# Autodesk Inventor assembly: AssemblyGefreesdBasev2
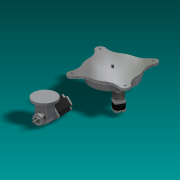
[picture p0: Inventor's stored thumbnail of the model, 180x180]
Saved by Autodesk Inventor 2020.2 (Build 242310000, 310)
## iProperties
Created: 2020-05-18
Part Number: AssemblyGefreesdBasev2
Document SubType Name: Assembly
Designer: Svend
Author: Svend
## Documents named in this file (14)
- C:\Users\Svend\OneDrive\Documents\GitHub\BeerMinder\3D-model\Base (Axis 1)\gefreesd\AssemblyGefreesdBasev2.iam
- C:\Users\Svend\OneDrive\Documents\GitHub\BeerMinder\3D-model\subAssembly\Nema17MetGearbox.iam
- C:\Users\Svend\OneDrive\Documents\GitHub\BeerMinder\3D-model\gearbox\afstandsplaatje.ipt
- C:\Users\Svend\OneDrive\Documents\GitHub\BeerMinder\3D-model\bearings\Ball Bearing 608ZZ.ipt
- C:\Users\Svend\OneDrive\Documents\GitHub\BeerMinder\3D-model\pulleys\GT2 Timing Pulley 20T - 8mm as.ipt
- C:\Users\Svend\OneDrive\Documents\GitHub\BeerMinder\3D-model\pulleys\GT2 Timing Pulley 60T - 8mm as.ipt
- C:\Users\Svend\OneDrive\Documents\GitHub\BeerMinder\3D-model\pulleys\Tandriem20naar60T.ipt
- C:\Users\Svend\OneDrive\Documents\GitHub\BeerMinder\3D-model\Base (Axis 1)\AsBase.ipt
- C:\Users\Svend\OneDrive\Documents\Inventor\Content Center Files\R2020\en-US\ISO 7380-1\ISO 7380-1 - M4 x 16.ipt
- C:\Users\Svend\OneDrive\Documents\GitHub\BeerMinder\3D-model\Base (Axis 1)\bevestiging axis 2.ipt
- C:\Users\Svend\OneDrive\Documents\GitHub\BeerMinder\3D-model\subAssembly\Nema23MetGearbox.iam
- C:\Users\Svend\OneDrive\Documents\GitHub\BeerMinder\3D-model\Base (Axis 1)\gefreesd\base bovenkant v2.ipt
- C:\Users\Svend\OneDrive\Documents\GitHub\BeerMinder\3D-model\Base (Axis 1)\gefreesd\kogel.ipt
- C:\Users\Svend\OneDrive\Documents\GitHub\BeerMinder\3D-model\Base (Axis 1)\gefreesd\onderkant base.ipt
## Components (55 placed, 13 different names)
1. base bovenkant v2:1 — Mate:6, Mate:20, Mate:7, Mate:29, Mate:33, Mate:34, Mate:35, Mate:36, Mate:41, Mate:42, Mate:43, Flush:5, Mate:45
2. Nema17MetGearbox:1 [sub-assembly] — Mate:3, Mate:4, Mate:5, Mate:20, Mate:13, Mate:28, Mate:30, Mate:31, Mate:32
3. afstandsplaatje:1 — Mate:3, Mate:4, Mate:5, Mate:6
4. Ball Bearing 608ZZ:1 — Mate:7, Mate:17, Flush:5
5. GT2 Timing Pulley 20T - 8mm as:1 — Mate:13, Flush:4, Mate:15, Mate:16
6. GT2 Timing Pulley 60T - 8mm as:1 — Mate:11, Mate:12, Flush:4, Mate:14, Mate:40, Mate:41
7. Ball Bearing 608ZZ:2 — Mate:11, Mate:12, Mate:44
8. Tandriem20naar60T:1 — Mate:14, Mate:15, Mate:16
9. AsBase:1 — Mate:17, Mate:40
10. ISO 7380-1 M4 x 16:1 — Mate:28, Mate:29
11. ISO 7380-1 M4 x 16:2 — Mate:30, Mate:35
12. ISO 7380-1 M4 x 16:3 — Mate:32, Mate:34
13. ISO 7380-1 M4 x 16:4 — Mate:31, Mate:33
14. bevestiging axis 2:1 — Mate:36, Mate:38, Mate:39
15. Nema23MetGearbox:1 [sub-assembly] — Mate:38, Mate:39
16. onderkant base:1 — Mate:44, Mate:45
17. kogel:1 — Mate:42, Mate:43
18. kogel:2
19. kogel:3
20. kogel:4
21. kogel:5
22. kogel:6
23. kogel:7
24. kogel:8
25. kogel:9
26. kogel:10
27. kogel:11
28. kogel:12
29. kogel:13
30. kogel:14
31. kogel:15
32. kogel:16
33. kogel:17
34. kogel:18
35. kogel:19
36. kogel:20
37. kogel:21
38. kogel:22
39. kogel:23
40. kogel:24
41. kogel:25
42. kogel:26
43. kogel:27
44. kogel:28
45. kogel:29
46. kogel:30
47. kogel:31
48. kogel:32
49. kogel:33
50. kogel:34
51. kogel:35
52. kogel:36
53. kogel:37
54. kogel:38
55. kogel:39
## Component patterns: (39 elements, first: kogel:1)
## Relationships (32: Mate 30, Flush 2)
- Mate:3: Nema17MetGearbox:1 ↔ afstandsplaatje:1
- Mate:4: Nema17MetGearbox:1 ↔ afstandsplaatje:1
- Mate:5: Nema17MetGearbox:1 ↔ afstandsplaatje:1
- Mate:6: base bovenkant v2:1 ↔ afstandsplaatje:1
- Mate:20: base bovenkant v2:1 ↔ Nema17MetGearbox:1
- Mate:7: base bovenkant v2:1 ↔ Ball Bearing 608ZZ:1
- Mate:11: GT2 Timing Pulley 60T - 8mm as:1 ↔ Ball Bearing 608ZZ:2
- Mate:12: GT2 Timing Pulley 60T - 8mm as:1 ↔ Ball Bearing 608ZZ:2
- Mate:13: Nema17MetGearbox:1 ↔ GT2 Timing Pulley 20T - 8mm as:1
- Flush:4: GT2 Timing Pulley 20T - 8mm as:1 ↔ GT2 Timing Pulley 60T - 8mm as:1
- Mate:14: GT2 Timing Pulley 60T - 8mm as:1 ↔ Tandriem20naar60T:1
- Mate:15: GT2 Timing Pulley 20T - 8mm as:1 ↔ Tandriem20naar60T:1
- Mate:16 (0.5 mm): GT2 Timing Pulley 20T - 8mm as:1 ↔ Tandriem20naar60T:1
- Mate:17: Ball Bearing 608ZZ:1 ↔ AsBase:1
- Mate:28: Nema17MetGearbox:1 ↔ ISO 7380-1 M4 x 16:1
- Mate:29: base bovenkant v2:1 ↔ ISO 7380-1 M4 x 16:1
- Mate:30: Nema17MetGearbox:1 ↔ ISO 7380-1 M4 x 16:2
- Mate:31: Nema17MetGearbox:1 ↔ ISO 7380-1 M4 x 16:4
- Mate:32: Nema17MetGearbox:1 ↔ ISO 7380-1 M4 x 16:3
- Mate:33: base bovenkant v2:1 ↔ ISO 7380-1 M4 x 16:4
- Mate:34: base bovenkant v2:1 ↔ ISO 7380-1 M4 x 16:3
- Mate:35: base bovenkant v2:1 ↔ ISO 7380-1 M4 x 16:2
- Mate:36: base bovenkant v2:1 ↔ bevestiging axis 2:1
- Mate:38: bevestiging axis 2:1 ↔ Nema23MetGearbox:1
- Mate:39: bevestiging axis 2:1 ↔ Nema23MetGearbox:1
- Mate:40: GT2 Timing Pulley 60T - 8mm as:1 ↔ AsBase:1
- Mate:41 (2 mm): base bovenkant v2:1 ↔ GT2 Timing Pulley 60T - 8mm as:1
- Mate:42 (95 mm): base bovenkant v2:1 ↔ kogel:1
- Mate:43 (1 mm): base bovenkant v2:1 ↔ kogel:1
- Flush:5: base bovenkant v2:1 ↔ Ball Bearing 608ZZ:1
- Mate:44: Ball Bearing 608ZZ:2 ↔ onderkant base:1
- Mate:45 (1 mm): base bovenkant v2:1 ↔ onderkant base:1
